# Autodesk Inventor assembly: Inner Assembly
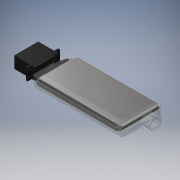
[picture p0: Inventor's stored thumbnail of the model, 180x180]
Saved by Autodesk Inventor 2018 (Build 220112000, 112)
## iProperties
Created: 2017-07-30
Part Number: Inner Assembly
Document SubType Name: Assembly
Designer: kurtis
Author: kurtis
## Documents named in this file (4)
- D:\Users\kurti\Git-Home\CAD\Sentry Camera V2\Inner Assembly.iam
- D:\Users\kurti\Git-Home\CAD\Sentry Camera V2\InnerGantry.ipt
- D:\Users\kurti\Git-Home\CAD\Sentry Camera V2\IphoneModel(Case).ipt
- D:\Users\kurti\Git-Home\CAD\Sentry Camera V2\FutabaS3003Rough.ipt
## Components (3 placed, 3 different names)
1. InnerGantry:1 — Mate:1, Mate:2, Mate:3, Mate:4, Mate:5, Flush:1
2. IphoneModel(Case):1 — Mate:1, Mate:2, Mate:3
3. FutabaS3003Rough:1 — Mate:4, Mate:5, Flush:1
## Relationships (6: Mate 5, Flush 1)
- Mate:1: InnerGantry:1 ↔ IphoneModel(Case):1
- Mate:2: InnerGantry:1 ↔ IphoneModel(Case):1
- Mate:3 (6 mm): InnerGantry:1 ↔ IphoneModel(Case):1
- Mate:4: InnerGantry:1 ↔ FutabaS3003Rough:1
- Mate:5: InnerGantry:1 ↔ FutabaS3003Rough:1
- Flush:1 (-11.75 mm): InnerGantry:1 ↔ FutabaS3003Rough:1
